# Autodesk Inventor assembly: printasm
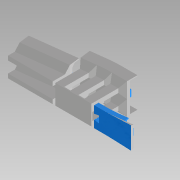
[picture p0: Inventor's stored thumbnail of the model, 180x180]
Saved by Autodesk Inventor 2021 (Build 250183000, 183)
## iProperties
Created: 2021-03-11
Part Number: printasm
Document SubType Name: Assembly
Designer: kumagai
Author: kumagai
## Documents named in this file (4)
- X:\Develop\CAD\PlaRails\Slope\printasm.iam
- X:\Develop\CAD\PlaRails\Slope\Slope_Middle_C.ipt
- X:\Develop\CAD\PlaRails\Slope\Slope_HighEnd_C.ipt
- X:\Develop\CAD\PlaRails\Slope\Slope_LowEnd_C.ipt
## Components (3 placed, 3 different names)
1. Slope_Middle_C:1 — フラッシュ:1, フラッシュ:2, フラッシュ:3, フラッシュ:4, メイト:1
2. Slope_HighEnd_C:1 — フラッシュ:1, フラッシュ:4, メイト:1, メイト:2
3. Slope_LowEnd_C:1 — フラッシュ:2, フラッシュ:3, メイト:2
## Relationships (6: Flush 4, Mate 2)
- フラッシュ:1 [Flush]: Slope_Middle_C:1 ↔ Slope_HighEnd_C:1
- フラッシュ:2 [Flush]: Slope_Middle_C:1 ↔ Slope_LowEnd_C:1
- フラッシュ:3 [Flush]: Slope_Middle_C:1 ↔ Slope_LowEnd_C:1
- フラッシュ:4 [Flush]: Slope_Middle_C:1 ↔ Slope_HighEnd_C:1
- メイト:1 [Mate] (5 mm): Slope_Middle_C:1 ↔ Slope_HighEnd_C:1
- メイト:2 [Mate] (5 mm): Slope_HighEnd_C:1 ↔ Slope_LowEnd_C:1
